# Autodesk Inventor assembly: ASY PRS 1200-90 Filter legs
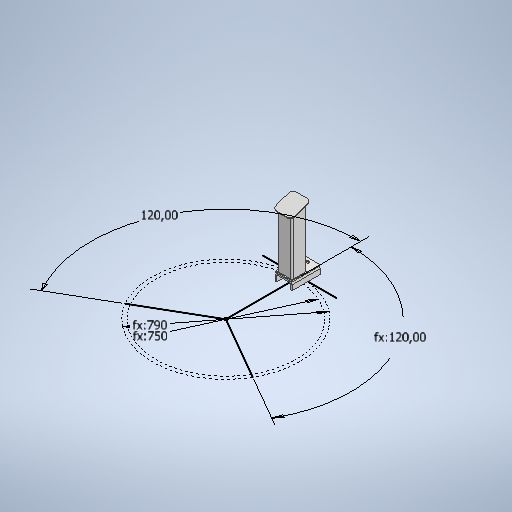
[picture p0: Inventor's stored thumbnail of the model, 512x512]
Saved by Autodesk Inventor 2025.4 (Build 294407000, 407)
## iProperties
Created: 2025-02-20
Part Number: ASY PRS 1200-90 Filter legs
Document SubType Name: Assembly
Designer: user
Mass: 20950.1 g
Surface Area: 14148.6 cm^2
Volume: 2651.55 cm^3
Density: 7.9011 g/cm^3
Author: user
## iProperties of the stored document MemberDocs/xFrdztucvNkfbe1veIejjgyne1b
Created: 2025-02-20
Part Number: ASY PRS 940-90 Filter legs
Document SubType Name: Assembly
Designer: user
Mass: 20950.1 g
Surface Area: 14148.6 cm^2
Volume: 2651.55 cm^3
Density: 7.9011 g/cm^3
Author: user
## Documents named in this file (6)
- C:\Users\admin\Documents\Inventor\PRS-Purovskii\Model\PRS-filter 1200\ASY PRS 1200-90 Filter legs.iam
- C:\Users\admin\Documents\Inventor\PRS-Purovskii\Model\PRS-filter 1200\PRS 940-92 Leg tube.ipt
- C:\Users\admin\Documents\Inventor\PRS-Purovskii\Model\PRS-filter 1200\PRS 940-93 leg sketch.ipt
- C:\Users\admin\Documents\Inventor\PRS-Purovskii\Model\PRS-filter 1200\PRS 940-94 leg plate for filter.ipt
- C:\Users\admin\Documents\Inventor\PRS-Purovskii\Model\PRS-filter 1200\PRS 940-95 leg floor plate.ipt
- C:\Users\admin\Documents\Inventor\PRS-Purovskii\Model\PRS-filter 1200\PRS 940-97 leg floor channel.ipt
## Components (6 placed, 6 different names)
1. PNS 1693 leg sketch.ipt:1 — Mate:6
2. PNS 1694 leg plate for filter.ipt:1 — Rigid:11
3. PNS 1695 leg floor plate.ipt:1 — Rigid:10, Mate:5, Flush:1
4. PNS 1696 leg floor pattern.ipt:1 — Mate:8, Flush:2, Flush:3
5. PNS 1692 Leg tube.ipt:2 — Mate:4, Mate:5, Flush:1, Mate:6, Rigid:11
6. PNS 1785 leg floor channel.ipt:1 — Rigid:10, Mate:1, Mate:2, Mate:8, Flush:2
## Relationships (11: Mate 6, Flush 3, WeldJoint 2)
- Rigid:10 [WeldJoint]: PNS 1695 leg floor plate.ipt:1 ↔ PNS 1785 leg floor channel.ipt:1
- Mate:1: PNS 1785 leg floor channel.ipt:1
- Mate:2: PNS 1785 leg floor channel.ipt:1
- Mate:4: PNS 1692 Leg tube.ipt:2
- Mate:5: PNS 1695 leg floor plate.ipt:1 ↔ PNS 1692 Leg tube.ipt:2
- Flush:1 (5 mm): PNS 1695 leg floor plate.ipt:1 ↔ PNS 1692 Leg tube.ipt:2
- Mate:6: PNS 1693 leg sketch.ipt:1 ↔ PNS 1692 Leg tube.ipt:2
- Mate:8: PNS 1696 leg floor pattern.ipt:1 ↔ PNS 1785 leg floor channel.ipt:1
- Flush:2: PNS 1696 leg floor pattern.ipt:1 ↔ PNS 1785 leg floor channel.ipt:1
- Flush:3: PNS 1696 leg floor pattern.ipt:1
- Rigid:11 [WeldJoint]: PNS 1694 leg plate for filter.ipt:1 ↔ PNS 1692 Leg tube.ipt:2
## Named parameters: Out_diam = 963 mm
